# Autodesk Inventor assembly: Assembly
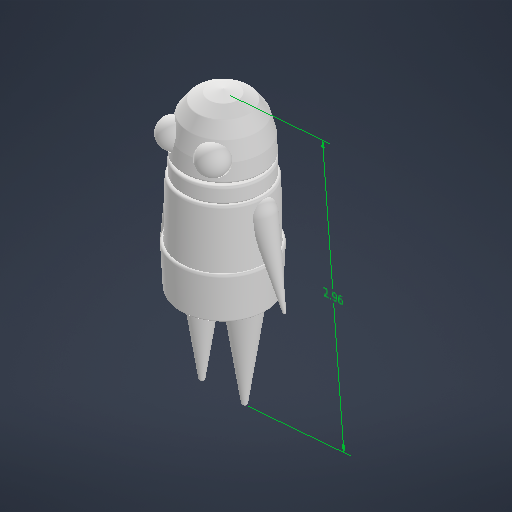
[picture p0: Inventor's stored thumbnail of the model, 512x512]
Saved by Autodesk Inventor 2025.2 (Build 292293000, 293)
## iProperties
Created: 2025-03-31
Part Number: Assembly
Document SubType Name: Assembly
Designer: mylap
Author: mylap
## Documents named in this file (7)
- C:\Users\mylap\Documents\Inventor\Repo Char\Assembly.iam
- C:\Users\mylap\Documents\Inventor\Repo Char\Body.ipt
- C:\Users\mylap\Documents\Inventor\Repo Char\Neck.ipt
- C:\Users\mylap\Documents\Inventor\Repo Char\Head.ipt
- C:\Users\mylap\Documents\Inventor\Repo Char\Eye.ipt
- C:\Users\mylap\Documents\Inventor\Repo Char\Arm.ipt
- C:\Users\mylap\Documents\Inventor\Repo Char\Leg.ipt
## Components (9 placed, 6 different names)
1. Body:1 — Insert:1, Mate:3, Mate:4, Mate:5, Mate:6
2. Neck:1 — Insert:1, Insert:2
3. Head:1 — Insert:2, Mate:1, Mate:2
4. Eye:1 — Mate:1
5. Eye:2 — Mate:2
6. Arm:2 — Mate:4
7. Arm:3 — Mate:3
8. Leg:1 — Mate:5
9. Leg:2 — Mate:6
## Relationships (8: Mate 6, Insert 2)
- Insert:1: Body:1 ↔ Neck:1
- Insert:2 (0.0794 mm): Neck:1 ↔ Head:1
- Mate:1: Head:1 ↔ Eye:1
- Mate:2: Head:1 ↔ Eye:2
- Mate:3: Body:1 ↔ Arm:3
- Mate:4: Body:1 ↔ Arm:2
- Mate:5: Body:1 ↔ Leg:1
- Mate:6: Body:1 ↔ Leg:2
